# Autodesk Inventor assembly: z stand
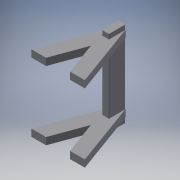
[picture p0: Inventor's stored thumbnail of the model, 180x180]
Saved by Autodesk Inventor 2019 (Build 230136000, 136)
## iProperties
Created: 2019-03-26
Part Number: z stand
Document SubType Name: Assembly
Designer: torba
Author: torba
## Documents named in this file (3)
- C:\Users\torba\Nextcloud\Projects\Inventor\Plasma 5x10\z stand.iam
- C:\Users\torba\Nextcloud\Projects\Inventor\Plasma 5x10\Wood 2x4x16.ipt
- C:\Users\torba\Nextcloud\Projects\Inventor\Plasma 5x10\2x4 leg stand.ipt
## Components (5 placed, 2 different names)
1. Wood 2x4x16:1 — Mate:1, Mate:2, Mate:3, Mate:4, Flush:3, Mate:6, Mate:7, Mate:9, Flush:4
2. 2x4 leg stand:1 — Flush:1, Mate:1, Flush:3, Mate:8, Mate:9
3. 2x4 leg stand:2 — Flush:1, Mate:4, Mate:8
4. 2x4 leg stand:3 — Flush:2, Mate:3, Mate:7, Flush:4
5. 2x4 leg stand:4 — Flush:2, Mate:2, Mate:6
## Relationships (12: Mate 8, Flush 4)
- Flush:1: 2x4 leg stand:1 ↔ 2x4 leg stand:2
- Flush:2: 2x4 leg stand:3 ↔ 2x4 leg stand:4
- Mate:1: Wood 2x4x16:1 ↔ 2x4 leg stand:1
- Mate:2: Wood 2x4x16:1 ↔ 2x4 leg stand:4
- Mate:3: Wood 2x4x16:1 ↔ 2x4 leg stand:3
- Mate:4: Wood 2x4x16:1 ↔ 2x4 leg stand:2
- Flush:3 (25.4 mm): Wood 2x4x16:1 ↔ 2x4 leg stand:1
- Mate:6: Wood 2x4x16:1 ↔ 2x4 leg stand:4
- Mate:7: Wood 2x4x16:1 ↔ 2x4 leg stand:3
- Mate:8: 2x4 leg stand:1 ↔ 2x4 leg stand:2
- Mate:9: Wood 2x4x16:1 ↔ 2x4 leg stand:1
- Flush:4 (25.4 mm): Wood 2x4x16:1 ↔ 2x4 leg stand:3
